# Autodesk Inventor assembly: Body Assembly
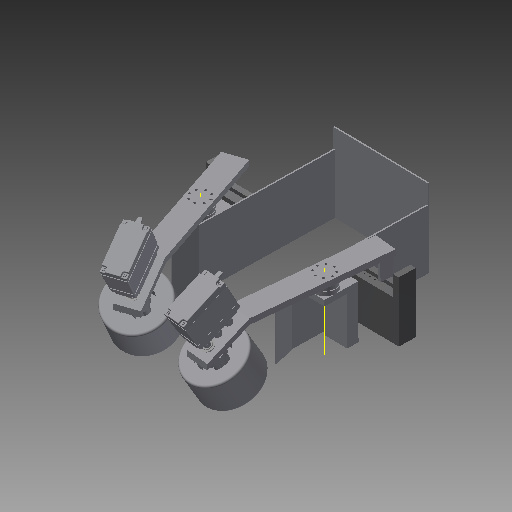
[picture p0: Inventor's stored thumbnail of the model, 512x512]
Saved by Autodesk Inventor 2019 (Build 230136000, 136)
## iProperties
Created: 2019-10-15
Part Number: Body Assembly
Document SubType Name: Assembly
Designer: User
Author: User
## Documents named in this file (17)
- C:\Robotics\2019-20_CAD\Collection\Body Assembly.iam
- C:\Robotics\2019-20_CAD\Collection\U-Part Gen 2.ipt
- C:\Robotics\COTSParts\Actobotics\545 parts\545364 assembly.ipt
- C:\Robotics\2019-20_CAD\Collection\wheel arm stand off.ipt
- C:\Robotics\2019-20_CAD\Collection\arm assembaly.iam
- C:\Robotics\COTSParts\Vex\2-Wire_Motor_393_276-2177.iam
- C:\Robotics\COTSParts\Wheels\2.5inFoamWheel250TMD.ipt
- C:\Robotics\2019-20_CAD\Collection\vex motor adaptor to tetrix.ipt
- C:\Robotics\COTSParts\Bearings - AndyMark\Bearing 250 ID 500 OD flanged.ipt
- C:\Robotics\COTSParts\Actobotics\545 parts\545364 assembly_MIR.ipt
- C:\Robotics\2019-20_CAD\Collection\wheel arm stand off_MIR.ipt
- C:\Robotics\2019-20_CAD\Collection\arm assembaly_MIR.iam
- C:\Robotics\COTSParts\Vex\2-Wire_Motor_393_276-2177_MIR.iam
- C:\Robotics\2019-20_CAD\Collection\vex motor adaptor to tetrix_MIR.ipt
- C:\Robotics\COTSParts\Wheels\2.5inFoamWheel250TMD_MIR.ipt
- C:\Robotics\COTSParts\Bearings - AndyMark\Bearing 250 ID 500 OD flanged_MIR1.ipt
- C:\Robotics\2019-20_CAD\Collection\Spring block.ipt
## Components (17 placed, 16 different names)
1. U-Part Gen 2:1 — Mate:23, Flush:10, Flush:25, Flush:27, Mate:57, Mate:58, Flush:29, Mate:60, Flush:30
2. 545364 assembly:2 — Mate:17, Mate:18, Mate:20
3. wheel arm stand off:2 — Mate:17, Mate:18, Mate:22, Mate:23, Flush:10, Flush:25, Flush:28, Mate:59
4. arm assembaly:1 [sub-assembly] — Mate:20, Mate:22, Mate:24, Mate:25, Mate:26, Mate:28, Mate:32
5. 2-Wire_Motor_393_276-2177:1 [sub-assembly] — Mate:24, Mate:25, Mate:26, Mate:27
6. vex motor adaptor to tetrix:1 — Mate:27, Mate:28, Mate:29, Insert:1, Mate:30, Mate:31
7. 2.5inFoamWheel250TMD:1 — Mate:29, Insert:1, Mate:30
8. Bearing 250 ID 500 OD flanged:1 — Mate:31, Mate:32
9. 545364 assembly_MIR:1 — Mate:41, Mate:42, Mate:44
10. wheel arm stand off_MIR:1 — Mate:41, Mate:42, Mate:43, Flush:27, Mate:57, Flush:28, Mate:61
11. arm assembaly_MIR:1 [sub-assembly] — Mate:43, Mate:44, Mate:45, Mate:46, Mate:47, Mate:48, Mate:52
12. 2-Wire_Motor_393_276-2177_MIR:1 [sub-assembly] — Mate:45, Mate:46, Mate:47, Mate:49
13. vex motor adaptor to tetrix_MIR:1 — Mate:48, Mate:49, Mate:50, Insert:2, Mate:51, Mate:53
14. 2.5inFoamWheel250TMD_MIR:1 — Mate:50, Insert:2, Mate:51
15. Bearing 250 ID 500 OD flanged_MIR1:1 — Mate:52, Mate:53
16. Spring block:1 — Mate:58, Mate:59, Flush:29
17. Spring block:2 — Mate:60, Flush:30, Mate:61
## Relationships (40: Mate 32, Flush 6, Insert 2)
- Mate:17: 545364 assembly:2 ↔ wheel arm stand off:2
- Mate:18: 545364 assembly:2 ↔ wheel arm stand off:2
- Mate:20: 545364 assembly:2 ↔ arm assembaly:1
- Mate:22: wheel arm stand off:2 ↔ arm assembaly:1
- Mate:23 (4.7625 mm): U-Part Gen 2:1 ↔ wheel arm stand off:2
- Flush:10 (-108.4072 mm): U-Part Gen 2:1 ↔ wheel arm stand off:2
- Mate:24: arm assembaly:1 ↔ 2-Wire_Motor_393_276-2177:1
- Mate:25: arm assembaly:1 ↔ 2-Wire_Motor_393_276-2177:1
- Mate:26: arm assembaly:1 ↔ 2-Wire_Motor_393_276-2177:1
- Mate:27: 2-Wire_Motor_393_276-2177:1 ↔ vex motor adaptor to tetrix:1
- Mate:28: arm assembaly:1 ↔ vex motor adaptor to tetrix:1
- Mate:29: vex motor adaptor to tetrix:1 ↔ 2.5inFoamWheel250TMD:1
- Insert:1: vex motor adaptor to tetrix:1 ↔ 2.5inFoamWheel250TMD:1
- Mate:30: vex motor adaptor to tetrix:1 ↔ 2.5inFoamWheel250TMD:1
- Mate:31: vex motor adaptor to tetrix:1 ↔ Bearing 250 ID 500 OD flanged:1
- Mate:32: arm assembaly:1 ↔ Bearing 250 ID 500 OD flanged:1
- Mate:41: 545364 assembly_MIR:1 ↔ wheel arm stand off_MIR:1
- Mate:42: 545364 assembly_MIR:1 ↔ wheel arm stand off_MIR:1
- Mate:43: wheel arm stand off_MIR:1 ↔ arm assembaly_MIR:1
- Mate:44: 545364 assembly_MIR:1 ↔ arm assembaly_MIR:1
- Mate:45: arm assembaly_MIR:1 ↔ 2-Wire_Motor_393_276-2177_MIR:1
- Mate:46: arm assembaly_MIR:1 ↔ 2-Wire_Motor_393_276-2177_MIR:1
- Mate:47: arm assembaly_MIR:1 ↔ 2-Wire_Motor_393_276-2177_MIR:1
- Mate:48: arm assembaly_MIR:1 ↔ vex motor adaptor to tetrix_MIR:1
- Mate:49: 2-Wire_Motor_393_276-2177_MIR:1 ↔ vex motor adaptor to tetrix_MIR:1
- Mate:50: vex motor adaptor to tetrix_MIR:1 ↔ 2.5inFoamWheel250TMD_MIR:1
- Insert:2: vex motor adaptor to tetrix_MIR:1 ↔ 2.5inFoamWheel250TMD_MIR:1
- Mate:51: vex motor adaptor to tetrix_MIR:1 ↔ 2.5inFoamWheel250TMD_MIR:1
- Mate:52: arm assembaly_MIR:1 ↔ Bearing 250 ID 500 OD flanged_MIR1:1
- Mate:53: vex motor adaptor to tetrix_MIR:1 ↔ Bearing 250 ID 500 OD flanged_MIR1:1
- Flush:25: U-Part Gen 2:1 ↔ wheel arm stand off:2
- Flush:27: U-Part Gen 2:1 ↔ wheel arm stand off_MIR:1
- Mate:57 (4.7625 mm): U-Part Gen 2:1 ↔ wheel arm stand off_MIR:1
- Flush:28: wheel arm stand off:2 ↔ wheel arm stand off_MIR:1
- Mate:58: U-Part Gen 2:1 ↔ Spring block:1
- Mate:59 (19.05 mm): wheel arm stand off:2 ↔ Spring block:1
- Flush:29: U-Part Gen 2:1 ↔ Spring block:1
- Mate:60: U-Part Gen 2:1 ↔ Spring block:2
- Flush:30: U-Part Gen 2:1 ↔ Spring block:2
- Mate:61 (19.05 mm): wheel arm stand off_MIR:1 ↔ Spring block:2
